# Autodesk Inventor assembly: Base Assembly rotated motors
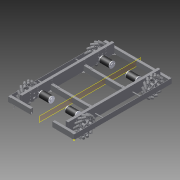
[picture p0: Inventor's stored thumbnail of the model, 180x180]
Saved by Autodesk Inventor 2015 (Build 190159000, 159)
## iProperties
Created: 2015-01-14
Part Number: Base Assembly rotated motors
Document SubType Name: Assembly
Designer: chapale16
Author: chapale16
## Documents named in this file (19)
- \\lhssvr02\Homedirs\Robotics Club\CAD Model 2015\CDR prep\Frame\Base Assembly rotated motors.iam
- \\lhssvr02\Homedirs\Robotics Club\CAD Model 2015\CDR prep\Frame\Frame front-back.ipt
- \\lhssvr02\Homedirs\Robotics Club\CAD Model 2015\Parts Folder\Wheels\Right Vex Mec Wheel.iam
- \\lhssvr02\Homedirs\Robotics Club\CAD Model 2015\CDR prep\Frame\Bumpers.ipt
- \\lhssvr02\Homedirs\Robotics Club\CAD Model 2015\Parts Folder\Wheels\Right Vex Mec Wheel_MIR.iam
- \\lhssvr02\Homedirs\Robotics Club\CAD Model 2015\Parts Folder\Wheels\Right Vex Mec Wheel_MIR1.iam
- \\lhssvr02\Homedirs\Robotics Club\CAD Model 2015\Parts Folder\Wheels\Right Vex Mec Wheel_MIR_MIR.iam
- \\lhssvr02\Homedirs\Robotics Club\CAD Model 2015\2x1 boxbeam 18 in.ipt
- \\lhssvr02\Homedirs\Robotics Club\CAD Model 2015\Modified Front Frame 27 in_MIR.ipt
- \\lhssvr02\Homedirs\Robotics Club\CAD Model 2015\Modified Front Frame 27 in_MIR_MIR.ipt
- \\lhssvr02\Homedirs\Robotics Club\CAD Model 2015\CDR prep\Frame\Standoffs Large.ipt
- \\lhssvr02\Homedirs\Robotics Club\CAD Model 2015\CDR prep\Frame\Standoffs Large_MIR.ipt
- \\lhssvr02\Homedirs\Robotics Club\CAD Model 2015\Box Beam Drive Base\Newest\Boxbeam.iam
- \\lhssvr02\Homedirs\Robotics Club\CAD Model 2015\Box Beam Drive Base\Newest\Boxbeam_MIR.iam
- \\lhssvr02\Homedirs\Robotics Club\CAD Model 2015\Parts Folder\Motors\Imported Components\MOT_CIM-Motor_217-2000.iam\FR801-001_CIM Motor Body.ipt
- \\lhssvr02\Homedirs\Robotics Club\CAD Model 2015\Parts Folder\Motors\Imported Components\MOT_CIM-Motor_217-2000.iam\FR801-001_CIM Motor Body_MIR.ipt
- \\lhssvr02\Homedirs\Robotics Club\CAD Model 2015\T-gusset.ipt
- \\lhssvr02\Homedirs\Robotics Club\CAD Model 2015\L-Gusset.ipt
- H:\Junior\c channel gusset.ipt
## Components (34 placed, 18 different names)
1. Frame front-back:2 — Mate:6, Flush:9, Mate:7, Mate:46, Mate:73, Mate:74, Flush:37, Flush:39
2. Right Vex Mec Wheel:2 [sub-assembly] — Mate:11
3. Bumpers:1 — Mate:6, Flush:9, Mate:7, Mate:13, Flush:12, Mate:14
4. Bumpers:2 — Mate:11, Mate:43, Mate:44
5. Right Vex Mec Wheel_MIR:1 [sub-assembly]
6. Right Vex Mec Wheel_MIR1:1 [sub-assembly]
7. Right Vex Mec Wheel_MIR_MIR:1 [sub-assembly]
8. 2x1 boxbeam 18 in:1 — Mate:45, Mate:64, Flush:34, Mate:66, Flush:35, Flush:44, Flush:50
9. Modified Front Frame 27 in_MIR:2 — Mate:13, Flush:12, Mate:14, Flush:13, Flush:18, Mate:70, Flush:47
10. Modified Front Frame 27 in_MIR_MIR:1 — Mate:77, Flush:45
11. Standoffs Large:1 — Mate:43
12. Standoffs Large:2 — Mate:44
13. Standoffs Large_MIR:1
14. Standoffs Large_MIR:2
15. Boxbeam:1 [sub-assembly] — Mate:45, Mate:46, Flush:13, Mate:47, Mate:48, Mate:49, Mate:50, Mate:63, Mate:65, Mate:71, Mate:72, Flush:38, Flush:48, Flush:49, Flush:51
16. Boxbeam_MIR:1 [sub-assembly] — Flush:17, Mate:54, Mate:67, Mate:68, Mate:75, Mate:76, Flush:40, Flush:41, Flush:43, Flush:46
17. FR801-001_CIM Motor Body:1 — Mate:47, Mate:48
18. FR801-001_CIM Motor Body:2 — Mate:49, Mate:50
19. FR801-001_CIM Motor Body_MIR:1
20. FR801-001_CIM Motor Body_MIR:2
21. 2x1 boxbeam 18 in:2 — Flush:17, Mate:54, Flush:18, Mate:62, Flush:33, Mate:69, Flush:36, Flush:42, Flush:52
22. L-Gusset:1 — Mate:62, Mate:63, Flush:33
23. L-Gusset:2 — Mate:64, Mate:65, Flush:34
24. L-Gusset:3 — Mate:68, Mate:69, Flush:36
25. L-Gusset:4 — Mate:66, Mate:67, Flush:35
26. T-gusset:1 — Mate:70, Flush:47, Flush:48
27. T-gusset:2 — Mate:71, Flush:49, Flush:50
28. T-gusset:3 — Mate:72, Flush:51, Flush:52
29. T-gusset:4 — Mate:73, Flush:37, Flush:38
30. T-gusset:5 — Mate:77, Flush:45, Flush:46
31. T-gusset:6 — Mate:76, Flush:43, Flush:44
32. T-gusset:7 — Mate:75, Flush:41, Flush:42
33. T-gusset:8 — Mate:74, Flush:39, Flush:40
34. c channel gusset:1
## Relationships (55: Mate 30, Flush 25)
- Mate:6: Frame front-back:2 ↔ Bumpers:1
- Flush:9: Frame front-back:2 ↔ Bumpers:1
- Mate:7: Frame front-back:2 ↔ Bumpers:1
- Mate:11 (22.86 mm): Right Vex Mec Wheel:2 ↔ Bumpers:2
- Mate:13: Bumpers:1 ↔ Modified Front Frame 27 in_MIR:2
- Flush:12: Bumpers:1 ↔ Modified Front Frame 27 in_MIR:2
- Mate:14: Bumpers:1 ↔ Modified Front Frame 27 in_MIR:2
- Mate:43: Bumpers:2 ↔ Standoffs Large:1
- Mate:44: Bumpers:2 ↔ Standoffs Large:2
- Mate:45: 2x1 boxbeam 18 in:1 ↔ Boxbeam:1
- Mate:46: Frame front-back:2 ↔ Boxbeam:1
- Flush:13: Modified Front Frame 27 in_MIR:2 ↔ Boxbeam:1
- Mate:47: Boxbeam:1 ↔ FR801-001_CIM Motor Body:1
- Mate:48: Boxbeam:1 ↔ FR801-001_CIM Motor Body:1
- Mate:49: Boxbeam:1 ↔ FR801-001_CIM Motor Body:2
- Mate:50: Boxbeam:1 ↔ FR801-001_CIM Motor Body:2
- Flush:17: Boxbeam_MIR:1 ↔ 2x1 boxbeam 18 in:2
- Mate:54: Boxbeam_MIR:1 ↔ 2x1 boxbeam 18 in:2
- Flush:18 (668.3502 mm): Modified Front Frame 27 in_MIR:2 ↔ 2x1 boxbeam 18 in:2
- Mate:62: 2x1 boxbeam 18 in:2 ↔ L-Gusset:1
- Mate:63: Boxbeam:1 ↔ L-Gusset:1
- Flush:33: 2x1 boxbeam 18 in:2 ↔ L-Gusset:1
- Mate:64: 2x1 boxbeam 18 in:1 ↔ L-Gusset:2
- Mate:65: Boxbeam:1 ↔ L-Gusset:2
- Flush:34: 2x1 boxbeam 18 in:1 ↔ L-Gusset:2
- Mate:66: 2x1 boxbeam 18 in:1 ↔ L-Gusset:4
- Mate:67: Boxbeam_MIR:1 ↔ L-Gusset:4
- Flush:35: 2x1 boxbeam 18 in:1 ↔ L-Gusset:4
- Mate:68: Boxbeam_MIR:1 ↔ L-Gusset:3
- Mate:69: 2x1 boxbeam 18 in:2 ↔ L-Gusset:3
- Flush:36: 2x1 boxbeam 18 in:2 ↔ L-Gusset:3
- Mate:70: Modified Front Frame 27 in_MIR:2 ↔ T-gusset:1
- Mate:71: Boxbeam:1 ↔ T-gusset:2
- Mate:72: Boxbeam:1 ↔ T-gusset:3
- Mate:73: Frame front-back:2 ↔ T-gusset:4
- Mate:74: Frame front-back:2 ↔ T-gusset:8
- Mate:75: Boxbeam_MIR:1 ↔ T-gusset:7
- Mate:76: Boxbeam_MIR:1 ↔ T-gusset:6
- Mate:77: Modified Front Frame 27 in_MIR_MIR:1 ↔ T-gusset:5
- Flush:37: Frame front-back:2 ↔ T-gusset:4
- Flush:38: Boxbeam:1 ↔ T-gusset:4
- Flush:39: Frame front-back:2 ↔ T-gusset:8
- Flush:40: Boxbeam_MIR:1 ↔ T-gusset:8
- Flush:41: Boxbeam_MIR:1 ↔ T-gusset:7
- Flush:42: 2x1 boxbeam 18 in:2 ↔ T-gusset:7
- Flush:43: Boxbeam_MIR:1 ↔ T-gusset:6
- Flush:44: 2x1 boxbeam 18 in:1 ↔ T-gusset:6
- Flush:45: Modified Front Frame 27 in_MIR_MIR:1 ↔ T-gusset:5
- Flush:46: Boxbeam_MIR:1 ↔ T-gusset:5
- Flush:47: Modified Front Frame 27 in_MIR:2 ↔ T-gusset:1
- Flush:48: Boxbeam:1 ↔ T-gusset:1
- Flush:49: Boxbeam:1 ↔ T-gusset:2
- Flush:50: 2x1 boxbeam 18 in:1 ↔ T-gusset:2
- Flush:51: Boxbeam:1 ↔ T-gusset:3
- Flush:52: 2x1 boxbeam 18 in:2 ↔ T-gusset:3
